# Autodesk Inventor assembly: korp
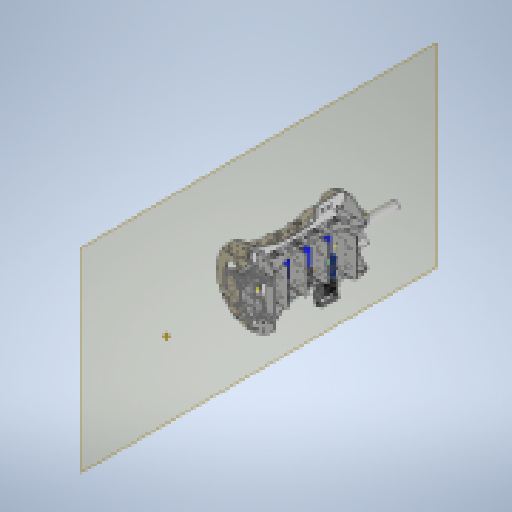
[picture p0: Inventor's stored thumbnail of the model, 512x512]
Saved by Autodesk Inventor 2023.1 (Build 271208000, 208)
## iProperties
Created: 2023-03-13
Part Number: korp
Document SubType Name: Assembly
Designer: User
Author: User
## Documents named in this file (34)
- C:\Users\DELL\reposGitHub\Cheburashka\Cheburashka_construction\korpus\korp.iam
- C:\Users\DELL\reposGitHub\Cheburashka\Cheburashka_construction\korpus\нижний эллипс тела.ipt
- C:\Users\DELL\reposGitHub\Cheburashka\Cheburashka_construction\korpus\грань тела.ipt
- C:\Users\DELL\reposGitHub\Cheburashka\Cheburashka_construction\korpus\верхний эллипс туловища.ipt
- C:\Users\DELL\reposGitHub\Cheburashka\Cheburashka_construction\korpus\Servo.ipt
- C:\Users\DELL\reposGitHub\Cheburashka\Cheburashka_construction\korpus\Pitsco Education-739028.ipt
- C:\Users\DELL\reposGitHub\Cheburashka\Cheburashka_construction\korpus\трубка.ipt
- C:\Users\DELL\reposGitHub\Cheburashka\Cheburashka_construction\korpus\Prostavka.ipt
- C:\Users\DELL\reposGitHub\Cheburashka\Cheburashka_construction\korpus\att_pin.ipt
- C:\Users\DELL\reposGitHub\Cheburashka\Cheburashka_construction\platform\KRAVT_holder_2 (1).ipt
- C:\Users\DELL\reposGitHub\Cheburashka\Cheburashka_construction\korpus\ребро.ipt
- C:\Users\DELL\reposGitHub\Cheburashka\Cheburashka_construction\korpus\ребро_MIR.ipt
- C:\Users\DELL\reposGitHub\Cheburashka\Cheburashka_construction\korpus\креп.ipt
- C:\Users\DELL\reposGitHub\Cheburashka\Cheburashka_construction\korpus\ребро0.5.ipt
- C:\Users\DELL\reposGitHub\Cheburashka\Cheburashka_construction\korpus\стабилизатор.ipt
- C:\Users\DELL\reposGitHub\Cheburashka\Cheburashka_construction\korpus\ограничитель.ipt
- C:\Users\DELL\reposGitHub\Cheburashka\Cheburashka_construction\korpus\ребро0.5_MIR3.ipt
- C:\Users\DELL\reposGitHub\Cheburashka\Cheburashka_construction\korpus\фанера.ipt
- C:\Users\DELL\reposGitHub\Cheburashka\Cheburashka_construction\korpus\ограничитель_MIR.ipt
- C:\Users\DELL\reposGitHub\Cheburashka\Cheburashka_construction\korpus\палка.ipt
- C:\Users\DELL\reposGitHub\Cheburashka\Cheburashka_construction\korpus\креп_MIR2.ipt
- C:\Users\DELL\reposGitHub\Cheburashka\Cheburashka_construction\korpus\палка_MIR.ipt
- C:\Users\DELL\reposGitHub\Cheburashka\Cheburashka_construction\korpus\raspberry-pi-4-model-b-1.snapshot.3\Raspberry Pi 4 Model B.iam
- C:\Users\DELL\reposGitHub\Cheburashka\Cheburashka_construction\korpus\arduino-mega-2650-1.snapshot.2\arduino MEGA2650.iam
- C:\Users\DELL\reposGitHub\Cheburashka\Cheburashka_construction\korpus\acc2.ipt
- C:\Users\DELL\reposGitHub\Cheburashka\Cheburashka_construction\korpus\acc1.ipt
- \\sch239.net\UserHomes\Students\other\baranovaem\Inventor\DS3240_Servomotor 40Kg 4.8-6.8v.ipt
- C:\Users\DELL\reposGitHub\Cheburashka\Cheburashka_construction\face\лицо\Pitsco Education-739086.iam
- C:\Users\DELL\reposGitHub\Cheburashka\Cheburashka_construction\face\лицо\креп_подш.ipt
- C:\Users\DELL\reposGitHub\Cheburashka\Cheburashka_construction\face\лицо\подшипник.ipt
- C:\Users\DELL\reposGitHub\Cheburashka\Cheburashka_construction\face\лицо\мини_подшипник.ipt
- C:\Users\DELL\reposGitHub\Cheburashka\Cheburashka_construction\face\лицо\ось_мини_подшипника.ipt
- C:\Users\DELL\reposGitHub\Cheburashka\Cheburashka_construction\face\лицо\креп_сервы.ipt
- C:\Users\DELL\reposGitHub\Cheburashka\Cheburashka_construction\korpus\кроватка.ipt
## Components (65 placed, 33 different names)
1. нижний эллипс тела:1 — Совмещение:100, Совмещение:121, Совмещение:139, Совмещение:140, Совмещение:209, Совмещение:210
2. верхний эллипс туловища:1 — Совмещение:223, Совмещение:236, Совмещение:237, Совмещение:244, Совмещение:267
3. грань тела:1 — Совмещение:209, Совмещение:210, Совмещение:211, Совмещение:214, Совмещение:223, Совмещение:224, Совмещение:225, Совмещение:229, Совмещение:236, Совмещение:237
4. Pitsco Education-739028:1 — Совмещение:283, Совмещение:284
5. Prostavka:1 — Совмещение:244, Совмещение:279, Совмещение:282
6. att_pin:1 — Совмещение:257, Совмещение:258, Совмещение:283, Совмещение:284
7. KRAVT_holder_2 (1):1 — Совмещение:100
8. ребро:1 — Совмещение:184, Совмещение:264
9. ребро_MIR:1 — Совмещение:122, Совмещение:188, Совмещение:204
10. креп:1 — Совмещение:159, Совмещение:166, Совмещение:221, Совмещение:222
11. креп:2 — Совмещение:164, Совмещение:165
12. креп:3 — Совмещение:162, Совмещение:163
13. креп:4 — Совмещение:160, Совмещение:161, Совмещение:219, Совмещение:220
14. креп:5 — Совмещение:167, Совмещение:168
15. креп:6 — Совмещение:169, Совмещение:170, Совмещение:183, Совмещение:217, Совмещение:218
16. креп:7 — Совмещение:261, Совмещение:262, Совмещение:263, Совмещение:265, Совмещение:266
17. креп:8 — Совмещение:171, Совмещение:172
18. трубка:2 — Совмещение:267, Совмещение:271, Совмещение:274, Совмещение:276, Совмещение:279, Совмещение:297
19. ребро0.5:1 — Совмещение:121, Совмещение:122, Совмещение:126, Совмещение:128, Совмещение:129, Совмещение:130, Совмещение:132, Совмещение:133, Совмещение:135, Совмещение:136, Совмещение:138, Совмещение:186, Совмещение:187, Совмещение:189, Совмещение:190, Совмещение:191, Совмещение:192, Совмещение:193, Совмещение:194, Совмещение:195, Совмещение:196, Совмещение:197, Совмещение:198, Совмещение:199, Совмещение:200, Совмещение:201, Совмещение:202
20. стабилизатор:1
21. ребро0.5_MIR3:1 — Совмещение:139, Совмещение:140, Совмещение:159, Совмещение:160, Совмещение:161, Совмещение:162, Совмещение:163, Совмещение:164, Совмещение:165, Совмещение:166, Совмещение:167, Совмещение:168, Совмещение:169, Совмещение:170, Совмещение:171, Совмещение:172, Совмещение:261, Совмещение:262
22. ограничитель:1 — Совмещение:126, Совмещение:128, Совмещение:129, Совмещение:175
23. ограничитель:2 — Совмещение:130, Совмещение:132
24. ограничитель:3 — Совмещение:133, Совмещение:135
25. ограничитель:4 — Совмещение:136, Совмещение:138
26. фанера:1 — Совмещение:175, Совмещение:263
27. ограничитель_MIR:1
28. ограничитель_MIR:2
29. ограничитель_MIR:3
30. ограничитель_MIR:4
31. палка:1 — Совмещение:264, Совмещение:265, Совмещение:266
32. креп_MIR2:1 — Совмещение:199, Совмещение:200, Совмещение:203
33. креп_MIR2:2 — Совмещение:201, Совмещение:202
34. креп_MIR2:3 — Совмещение:197, Совмещение:198
35. креп_MIR2:4 — Совмещение:185, Совмещение:186, Совмещение:187
36. креп_MIR2:5 — Совмещение:195, Совмещение:196
37. креп_MIR2:6 — Совмещение:189, Совмещение:190
38. креп_MIR2:7 — Совмещение:180, Совмещение:181, Совмещение:182, Совмещение:191, Совмещение:192
39. креп_MIR2:8 — Совмещение:193, Совмещение:194
40. палка_MIR:1 — Совмещение:180, Совмещение:181, Совмещение:182
41. фанера:2 — Совмещение:183, Совмещение:184, Совмещение:212, Совмещение:213
42. фанера:3 — Совмещение:203, Совмещение:204
43. фанера:4 — Совмещение:185, Совмещение:188, Совмещение:215, Совмещение:216
44. Raspberry Pi 4 Model B:1 [sub-assembly] — Совмещение:212, Совмещение:213
45. arduino MEGA2650:1 [sub-assembly] — Совмещение:215, Совмещение:216
46. стабилизатор:2 — Совмещение:214
47. стабилизатор:3 — Совмещение:211
48. палка:2 — Совмещение:219, Совмещение:220
49. палка:3 — Совмещение:221, Совмещение:222
50. палка:4 — Совмещение:217, Совмещение:218
51. Servo:5 — Совмещение:224, Совмещение:225, Совмещение:227, Совмещение:228
52. acc2:1 — Совмещение:227, Совмещение:228
53. acc1:1 — Совмещение:229
54. DS3240_Servomotor 40Kg 4.8-6.8v:2 — Совмещение:257, Совмещение:258, Совмещение:293, Совмещение:294, Совмещение:295, Совмещение:296
55. Pitsco Education-739086:1 [sub-assembly] — Совмещение:271, Совмещение:274, Совмещение:280, Совмещение:282, Совмещение:286, Совмещение:288, Совмещение:298
56. креп_подш:1 — Совмещение:287, Совмещение:288, Совмещение:291, Касательность:2
57. подшипник:1 — Совмещение:276, Совмещение:280, Совмещение:285, Совмещение:287
58. креп_подш:2 — Совмещение:285, Совмещение:286, Касательность:1
59. мини_подшипник:1 — Совмещение:289
60. ось_мини_подшипника:1 — Совмещение:289, Касательность:1
61. мини_подшипник:2 — Совмещение:292
62. ось_мини_подшипника:2 — Совмещение:291, Касательность:2, Совмещение:292
63. креп_сервы:1 — Совмещение:295, Совмещение:296
64. креп_сервы:2 — Совмещение:293, Совмещение:294
65. кроватка:1 — Совмещение:297, Совмещение:298
## Relationships (110: Mate 107, Tangent 2, Angle 1)
- Совмещение:100 [Mate]: нижний эллипс тела:1 ↔ KRAVT_holder_2 (1):1
- Совмещение:121 [Mate]: нижний эллипс тела:1 ↔ ребро0.5:1
- Совмещение:122 [Mate]: ребро_MIR:1 ↔ ребро0.5:1
- Совмещение:126 [Mate]: ребро0.5:1 ↔ ограничитель:1
- Совмещение:128 [Mate]: ребро0.5:1 ↔ ограничитель:1
- Совмещение:129 [Mate]: ребро0.5:1 ↔ ограничитель:1
- Совмещение:130 [Mate]: ребро0.5:1 ↔ ограничитель:2
- Совмещение:132 [Mate]: ребро0.5:1 ↔ ограничитель:2
- Совмещение:133 [Mate]: ребро0.5:1 ↔ ограничитель:3
- Совмещение:135 [Mate]: ребро0.5:1 ↔ ограничитель:3
- Совмещение:136 [Mate]: ребро0.5:1 ↔ ограничитель:4
- Совмещение:138 [Mate]: ребро0.5:1 ↔ ограничитель:4
- Совмещение:139 [Mate]: нижний эллипс тела:1 ↔ ребро0.5_MIR3:1
- Совмещение:140 [Mate]: нижний эллипс тела:1 ↔ ребро0.5_MIR3:1
- Совмещение:159 [Mate]: креп:1 ↔ ребро0.5_MIR3:1
- Совмещение:160 [Mate]: креп:4 ↔ ребро0.5_MIR3:1
- Совмещение:161 [Mate]: креп:4 ↔ ребро0.5_MIR3:1
- Совмещение:162 [Mate]: креп:3 ↔ ребро0.5_MIR3:1
- Совмещение:163 [Mate]: креп:3 ↔ ребро0.5_MIR3:1
- Совмещение:164 [Mate]: креп:2 ↔ ребро0.5_MIR3:1
- Совмещение:165 [Mate]: креп:2 ↔ ребро0.5_MIR3:1
- Совмещение:166 [Mate]: креп:1 ↔ ребро0.5_MIR3:1
- Совмещение:167 [Mate]: креп:5 ↔ ребро0.5_MIR3:1
- Совмещение:168 [Mate]: креп:5 ↔ ребро0.5_MIR3:1
- Совмещение:169 [Mate]: креп:6 ↔ ребро0.5_MIR3:1
- Совмещение:170 [Mate]: креп:6 ↔ ребро0.5_MIR3:1
- Совмещение:171 [Mate]: креп:8 ↔ ребро0.5_MIR3:1
- Совмещение:172 [Mate]: креп:8 ↔ ребро0.5_MIR3:1
- Совмещение:175 [Mate]: ограничитель:1 ↔ фанера:1
- Совмещение:180 [Mate]: креп_MIR2:7 ↔ палка_MIR:1
- Совмещение:181 [Mate]: креп_MIR2:7 ↔ палка_MIR:1
- Совмещение:182 [Mate]: креп_MIR2:7 ↔ палка_MIR:1
- Совмещение:183 [Mate]: креп:6 ↔ фанера:2
- Совмещение:184 [Mate]: ребро:1 ↔ фанера:2
- Совмещение:185 [Mate]: креп_MIR2:4 ↔ фанера:4
- Совмещение:186 [Mate]: ребро0.5:1 ↔ креп_MIR2:4
- Совмещение:187 [Mate]: ребро0.5:1 ↔ креп_MIR2:4
- Совмещение:188 [Mate]: ребро_MIR:1 ↔ фанера:4
- Совмещение:189 [Mate]: ребро0.5:1 ↔ креп_MIR2:6
- Совмещение:190 [Mate]: ребро0.5:1 ↔ креп_MIR2:6
- Совмещение:191 [Mate]: ребро0.5:1 ↔ креп_MIR2:7
- Совмещение:192 [Mate]: ребро0.5:1 ↔ креп_MIR2:7
- Совмещение:193 [Mate]: ребро0.5:1 ↔ креп_MIR2:8
- Совмещение:194 [Mate]: ребро0.5:1 ↔ креп_MIR2:8
- Совмещение:195 [Mate]: ребро0.5:1 ↔ креп_MIR2:5
- Совмещение:196 [Mate]: ребро0.5:1 ↔ креп_MIR2:5
- Совмещение:197 [Mate]: ребро0.5:1 ↔ креп_MIR2:3
- Совмещение:198 [Mate]: ребро0.5:1 ↔ креп_MIR2:3
- Совмещение:199 [Mate]: ребро0.5:1 ↔ креп_MIR2:1
- Совмещение:200 [Mate]: ребро0.5:1 ↔ креп_MIR2:1
- Совмещение:201 [Mate]: ребро0.5:1 ↔ креп_MIR2:2
- Совмещение:202 [Mate]: ребро0.5:1 ↔ креп_MIR2:2
- Совмещение:203 [Mate]: креп_MIR2:1 ↔ фанера:3
- Совмещение:204 [Mate]: ребро_MIR:1 ↔ фанера:3
- Совмещение:209 [Mate]: нижний эллипс тела:1 ↔ грань тела:1
- Совмещение:210 [Mate]: нижний эллипс тела:1 ↔ грань тела:1
- Совмещение:211 [Mate]: грань тела:1 ↔ стабилизатор:3
- Совмещение:212 [Mate]: фанера:2 ↔ Raspberry Pi 4 Model B:1
- Совмещение:213 [Mate]: фанера:2 ↔ Raspberry Pi 4 Model B:1
- Совмещение:214 [Mate]: грань тела:1 ↔ стабилизатор:2
- Совмещение:215 [Mate]: фанера:4 ↔ arduino MEGA2650:1
- Совмещение:216 [Mate]: фанера:4 ↔ arduino MEGA2650:1
- Совмещение:217 [Mate]: креп:6 ↔ палка:4
- Совмещение:218 [Mate]: креп:6 ↔ палка:4
- Совмещение:219 [Mate]: креп:4 ↔ палка:2
- Совмещение:220 [Mate]: креп:4 ↔ палка:2
- Совмещение:221 [Mate]: креп:1 ↔ палка:3
- Совмещение:222 [Mate]: креп:1 ↔ палка:3
- Совмещение:223 [Mate]: верхний эллипс туловища:1 ↔ грань тела:1
- Совмещение:224 [Mate]: грань тела:1 ↔ Servo:5
- Совмещение:225 [Mate]: грань тела:1 ↔ Servo:5
- Совмещение:227 [Mate]: Servo:5 ↔ acc2:1
- Совмещение:228 [Mate]: Servo:5 ↔ acc2:1
- Совмещение:229 [Mate]: грань тела:1 ↔ acc1:1
- Совмещение:236 [Mate]: верхний эллипс туловища:1 ↔ грань тела:1
- Совмещение:237 [Mate]: верхний эллипс туловища:1 ↔ грань тела:1
- Совмещение:244 [Mate]: верхний эллипс туловища:1 ↔ Prostavka:1
- Совмещение:257 [Mate]: att_pin:1 ↔ DS3240_Servomotor 40Kg 4.8-6.8v:2
- Совмещение:258 [Mate]: att_pin:1 ↔ DS3240_Servomotor 40Kg 4.8-6.8v:2
- Угол:1 [Angle] (0 deg)
- Совмещение:261 [Mate]: креп:7 ↔ ребро0.5_MIR3:1
- Совмещение:262 [Mate]: креп:7 ↔ ребро0.5_MIR3:1
- Совмещение:263 [Mate]: креп:7 ↔ фанера:1
- Совмещение:264 [Mate]: ребро:1 ↔ палка:1
- Совмещение:265 [Mate]: креп:7 ↔ палка:1
- Совмещение:266 [Mate]: креп:7 ↔ палка:1
- Совмещение:267 [Mate]: верхний эллипс туловища:1 ↔ трубка:2
- Совмещение:271 [Mate]: трубка:2 ↔ Pitsco Education-739086:1
- Совмещение:274 [Mate]: трубка:2 ↔ Pitsco Education-739086:1
- Совмещение:276 [Mate]: трубка:2 ↔ подшипник:1
- Совмещение:279 [Mate]: Prostavka:1 ↔ трубка:2
- Совмещение:280 [Mate] (2 mm): Pitsco Education-739086:1 ↔ подшипник:1
- Совмещение:282 [Mate]: Prostavka:1 ↔ Pitsco Education-739086:1
- Совмещение:283 [Mate]: Pitsco Education-739028:1 ↔ att_pin:1
- Совмещение:284 [Mate]: Pitsco Education-739028:1 ↔ att_pin:1
- Совмещение:285 [Mate]: подшипник:1 ↔ креп_подш:2
- Совмещение:286 [Mate]: Pitsco Education-739086:1 ↔ креп_подш:2
- Совмещение:287 [Mate]: креп_подш:1 ↔ подшипник:1
- Совмещение:288 [Mate]: Pitsco Education-739086:1 ↔ креп_подш:1
- Совмещение:289 [Mate]: мини_подшипник:1 ↔ ось_мини_подшипника:1
- Касательность:1 [Tangent]: креп_подш:2 ↔ ось_мини_подшипника:1
- Совмещение:291 [Mate]: креп_подш:1 ↔ ось_мини_подшипника:2
- Касательность:2 [Tangent]: креп_подш:1 ↔ ось_мини_подшипника:2
- Совмещение:292 [Mate]: мини_подшипник:2 ↔ ось_мини_подшипника:2
- Совмещение:293 [Mate]: DS3240_Servomotor 40Kg 4.8-6.8v:2 ↔ креп_сервы:2
- Совмещение:294 [Mate]: DS3240_Servomotor 40Kg 4.8-6.8v:2 ↔ креп_сервы:2
- Совмещение:295 [Mate]: DS3240_Servomotor 40Kg 4.8-6.8v:2 ↔ креп_сервы:1
- Совмещение:296 [Mate]: DS3240_Servomotor 40Kg 4.8-6.8v:2 ↔ креп_сервы:1
- Совмещение:297 [Mate]: трубка:2 ↔ кроватка:1
- Совмещение:298 [Mate]: Pitsco Education-739086:1 ↔ кроватка:1
